# Autodesk Inventor assembly: !drivetrain
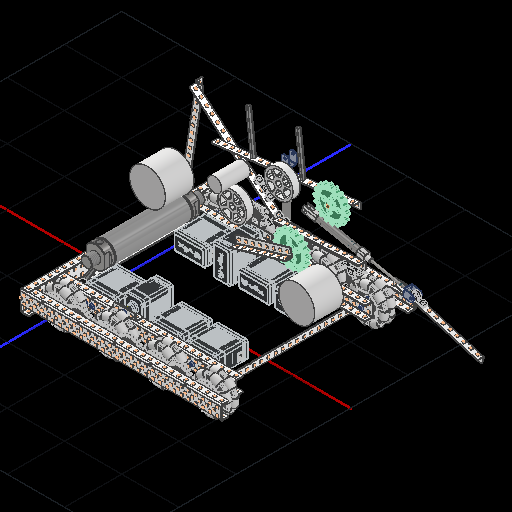
[picture p0: Inventor's stored thumbnail of the model, 512x512]
Saved by Autodesk Inventor 2025.2 (Build 292293000, 293)
## iProperties
Created: 2025-11-15
Part Number: !drivetrain
Document SubType Name: Assembly
Designer: cloudy
Author: cloudy
## Documents named in this file (43)
- C:\Users\cloudy\Documents\AURA_CAD\15\Drivetrain\!drivetrain.iam
- C:\Users\cloudy\Documents\AURA_CAD\15\Drivetrain\Wheels\Omni\2.75\2.75 Omni Assembly.iam
- C:\Users\cloudy\Documents\AURA_CAD\!lib\Structure\C Channel\Aluminum 1x2x1\Alu C 1x2x1x28.ipt
- C:\Users\cloudy\Documents\AURA_CAD\!lib\Structure\Hardware\Screw Steel - Star\SScrew Star Smooth 2.000.ipt
- C:\Users\cloudy\Documents\AURA_CAD\!lib\Structure\Hardware\Screw Steel - Star.ipt
- C:\Users\cloudy\Documents\AURA_CAD\!lib\Structure\Hardware\Nut Keps.ipt
- C:\Users\cloudy\Documents\AURA_CAD\!lib\Motion\Shaft LS\LS Pillow Bearing Block.ipt
- C:\Users\cloudy\Documents\AURA_CAD\!lib\Structure\C Channel\Aluminum 1x3x1 Half\Alu C Half 1x3x1x19.ipt
- C:\Users\cloudy\Documents\AURA_CAD\!lib\Structure\C Channel\Aluminum 1x2x1\Alu C 1x2x1x26.ipt
- C:\Users\cloudy\Documents\AURA_CAD\!lib\Structure\C Channel\Aluminum 1x3x1\Alu C 1x3x1x27.ipt
- C:\Users\cloudy\Documents\AURA_CAD\15\Drivetrain\Gears\26t_no_screwholes.ipt
- C:\Users\cloudy\Documents\AURA_CAD\!lib\Electronics\Motors with Screws\AluM-StarS.iam
- C:\Users\cloudy\Documents\AURA_CAD\!lib\Electronics\Motors with Screws.iam
- C:\Users\cloudy\Documents\AURA_CAD\15\Drivetrain\bearing_2 long.ipt
- C:\Users\cloudy\Documents\AURA_CAD\!lib\Motion\Spacers\Spacer Nylon .500 OD\NSpacer White .500 OD x .125.ipt
- C:\Users\cloudy\Documents\AURA_CAD\!lib\Motion\Spacers\Spacer Nylon .500 OD.ipt
- C:\Users\cloudy\Documents\AURA_CAD\!lib\Motion\Spacers\Spacer Nylon .375 OD\NSpacer .375 OD x .500.ipt
- C:\Users\cloudy\Documents\AURA_CAD\!lib\Motion\Spacers\Spacer Nylon .375 OD.ipt
- C:\Users\cloudy\Documents\AURA_CAD\!lib\Motion\Spacers\Spacer Nylon .375 OD\NSpacer .375 OD x .250.ipt
- C:\Users\cloudy\Documents\AURA_CAD\!lib\Motion\Shaft LS\Bearing Flat - Drilled.ipt
- C:\Users\cloudy\Documents\AURA_CAD\!lib\Motion\Shaft LS\Shaft Collar Metal\Shaft Collar No Screw.iam
- C:\Users\cloudy\Documents\AURA_CAD\!lib\Motion\Shaft LS\Shaft Collar Metal.iam
- C:\Users\cloudy\Documents\AURA_CAD\!lib\Structure\Standoff\Standoff 3.00.ipt
- C:\Users\cloudy\Documents\AURA_CAD\!lib\Structure\Standoff.ipt
- C:\Users\cloudy\Documents\AURA_CAD\!lib\Motion\Spacers\Spacer Nylon .375 OD\NSpacer .375 OD x .375.ipt
- C:\Users\cloudy\Documents\AURA_CAD\!lib\Motion\Spacers\Washer Steel\SWasher .375 OD x .062500.ipt
- C:\Users\cloudy\Documents\AURA_CAD\!lib\Motion\Spacers\Washer Steel.ipt
- C:\Users\cloudy\Documents\AURA_CAD\!lib\Structure\C Channel\Aluminum 1x3x1 Half\Alu C Half 1x3x1x3.ipt
- C:\Users\cloudy\Documents\AURA_CAD\!lib\Structure\C Channel\Aluminum 1x3x1 Half\Alu C Half 1x3x1x20.ipt
- C:\Users\cloudy\Documents\AURA_CAD\!lib\Motion\Pneumatics\Legacy - SMC Pneumatics\Double Acting Piston.iam
- C:\Users\cloudy\Documents\AURA_CAD\!lib\Motion\Pneumatics\Legacy - SMC Pneumatics\Cylinder Mount.ipt
- C:\Users\cloudy\Documents\AURA_CAD\!lib\Structure\C Channel\Aluminum 1x3x1 Half\Alu C Half 1x3x1x23.ipt
- C:\Users\cloudy\Documents\AURA_CAD\!lib\Structure\C Channel\Aluminum 1x3x1 Half\Alu C Half 1x3x1x15.ipt
- C:\Users\cloudy\Documents\AURA_CAD\!lib\Motion\Sprockets\9P Sprocket.iam
- C:\Users\cloudy\Documents\AURA_CAD\!lib\Motion\Sprockets\9P Sprocket\9P 18T Sprocket, Circle.iam
- C:\Users\cloudy\Documents\AURA_CAD\15\2.5in roller.ipt
- C:\Users\cloudy\Documents\AURA_CAD\!lib\Motion\Wheels\Flex Wheels\2.000 Flex Wheel\2.000 30A .500.ipt
- C:\Users\cloudy\Documents\AURA_CAD\!lib\Motion\Wheels\Flex Wheels\2.000 Flex Wheel.ipt
- C:\Users\cloudy\Documents\AURA_CAD\15\1 in roller.ipt
- C:\Users\cloudy\Documents\AURA_CAD\!lib\Motion\Pneumatics\Legacy - SMC Pneumatics\Reservoir.ipt
- C:\Users\cloudy\Documents\AURA_CAD\!lib\Structure\C Channel\Aluminum 1x3x1 Half\Alu C Half 1x3x1x8.ipt
- C:\Users\cloudy\Documents\AURA_CAD\!lib\Structure\C Channel\Aluminum 1x3x1 Half\Alu C Half 1x3x1x12.ipt
- C:\Users\cloudy\Documents\AURA_CAD\!lib\Structure\C Channel\Aluminum 1x3x1 Half\Alu C Half 1x3x1x2.ipt
## Components (111 placed, 33 different names)
1. Alu C 1x2x1x26:1 — Insert:10, Insert:19, Insert:20, Insert:23, Insert:26, Mate:18, Insert:36, Insert:40, Mate:22, Mate:23, Insert:41, Insert:42, Insert:43, Insert:47, Mate:24, Insert:51, Insert:67, Insert:90, Mate:37, Mate:38, Insert:102, Mate:44, Insert:112, Angle:1
2. 2.75 Omni Assembly:1 [sub-assembly] — Insert:45
3. Alu C 1x2x1x28:2 — Mate:17, Insert:33
4. Alu C 1x2x1x26:2 — Mate:14, Mate:18, Insert:31, Insert:93, Mate:39
5. SScrew Star Smooth 2.000:1 — Insert:10, Mate:26
6. 2.75 Omni Assembly:5 [sub-assembly] — Insert:46
7. SScrew Star Smooth 2.000:2 — Insert:20
8. 2.75 Omni Assembly:6 [sub-assembly] — Insert:23
9. SScrew Star Smooth 2.000:3 — Insert:19
10. 2.75 Omni Assembly:7 [sub-assembly] — Insert:44
11. Alu C Half 1x3x1x19:1 — Insert:26, Insert:31
12. Alu C 1x3x1x27:1 — Mate:14, Mate:15, Mate:16, Mate:17, Insert:32, Insert:33, Mate:34, Insert:72, Insert:108
13. 26t_no_screwholes:1 — Insert:52, Insert:56
14. 26t_no_screwholes:2 — Insert:53, Insert:55
15. 26t_no_screwholes:3 — Insert:54, Insert:57
16. Alu C 1x2x1x28:3 — Insert:32, Mate:26, Insert:52, Insert:53, Insert:54, Insert:58, Insert:59, Insert:60, Mate:27, Mate:28, Mate:29, Insert:61, Mate:30, Insert:62, Insert:63, Insert:64, Mate:31, Mate:32, Mate:33, Insert:130, Mate:57
17. AluM-StarS:1 [sub-assembly] — Insert:36, Mate:22
18. AluM-StarS:2 [sub-assembly] — Insert:40, Mate:23
19. AluM-StarS:3 [sub-assembly] — Insert:47, Mate:24
20. Nut Keps:1 — Insert:41, Insert:44
21. Nut Keps:2 — Insert:42, Insert:45
22. Nut Keps:3 — Insert:43, Insert:46
23. NSpacer White .500 OD x .125:2 — Insert:51
24. NSpacer .375 OD x .250:2 — Insert:56
25. NSpacer .375 OD x .250:3 — Insert:55
26. NSpacer .375 OD x .250:4 — Insert:57
27. bearing_2 long:3 — Insert:59, Mate:28
28. bearing_2 long:4 — Insert:61, Mate:30
29. bearing_2 long:5 — Insert:58, Mate:29
30. bearing_2 long:6 — Insert:60, Mate:27
31. Bearing Flat - Drilled:1 — Insert:62, Mate:33
32. Bearing Flat - Drilled:2 — Insert:64, Mate:31
33. Bearing Flat - Drilled:3 — Insert:63, Mate:32
34. Shaft Collar No Screw:1 [sub-assembly] — Insert:67, Mate:35, Insert:69
35. Shaft Collar No Screw:2 [sub-assembly] — Mate:34, Mate:35, Insert:68, Insert:74
36. Standoff 3.00:1 — Insert:70
37. NSpacer .375 OD x .500:5 — Insert:68
38. NSpacer .375 OD x .375:6 — Insert:69, Insert:70
39. NSpacer .375 OD x .500:7 — Insert:71, Insert:73
40. NSpacer .375 OD x .500:8 — Insert:71, Insert:72
41. SWasher .375 OD x .062500:1 — Insert:73
42. SWasher .375 OD x .062500:2 — Insert:74
43. 2.75 Omni Assembly:8 [sub-assembly] — Insert:76
44. SScrew Star Smooth 2.000:6
45. 2.75 Omni Assembly:9 [sub-assembly] — Insert:77
46. SScrew Star Smooth 2.000:7
47. 2.75 Omni Assembly:10 [sub-assembly]
48. SScrew Star Smooth 2.000:8
49. 2.75 Omni Assembly:11 [sub-assembly] — Insert:75
50. 26t_no_screwholes:4 — Insert:80
51. 26t_no_screwholes:5 — Insert:81
52. 26t_no_screwholes:6 — Insert:82
53. AluM-StarS:4 [sub-assembly]
54. AluM-StarS:5 [sub-assembly]
55. AluM-StarS:6 [sub-assembly]
56. Nut Keps:4 — Insert:75
57. Nut Keps:5 — Insert:76
58. Nut Keps:6 — Insert:77
59. NSpacer White .500 OD x .125:4
60. NSpacer .375 OD x .250:10 — Insert:80
61. NSpacer .375 OD x .250:11 — Insert:81
62. NSpacer .375 OD x .250:12 — Insert:82
63. bearing_2 long:7
64. bearing_2 long:8
65. bearing_2 long:9
66. bearing_2 long:10
67. Bearing Flat - Drilled:4
68. Bearing Flat - Drilled:5
69. Bearing Flat - Drilled:6
70. Shaft Collar No Screw:3 [sub-assembly] — Mate:36, Insert:86
71. Shaft Collar No Screw:4 [sub-assembly] — Mate:36, Insert:84, Insert:89
72. Standoff 3.00:2 — Insert:85
73. NSpacer .375 OD x .500:13 — Insert:84
74. NSpacer .375 OD x .375:14 — Insert:85, Insert:86
75. NSpacer .375 OD x .500:15 — Insert:87, Insert:88
76. NSpacer .375 OD x .500:16 — Insert:87
77. SWasher .375 OD x .062500:3 — Insert:88
78. SWasher .375 OD x .062500:4 — Insert:89
79. Alu C Half 1x3x1x3:1 — Insert:90, Mate:37, Insert:91
80. AluM-StarS:7 [sub-assembly] — Insert:91, Mate:38
81. Alu C Half 1x3x1x3:2 — Insert:92, Insert:93, Mate:39
82. AluM-StarS:8 [sub-assembly] — Insert:92
83. Alu C Half 1x3x1x23:1 — Mate:48, Insert:110, Insert:121, Mate:53, Insert:123, Mate:54, Insert:126, Mate:55, Mate:138
84. LS Pillow Bearing Block:2 — Insert:102, Mate:44
85. Shaft Collar No Screw:5 [sub-assembly] — Insert:108, Insert:109
86. Alu C Half 1x3x1x15:1 — Insert:109, Mate:48
87. Alu C Half 1x3x1x20:1 — Insert:110, Insert:111, Mate:51, Mate:52, Insert:115, Insert:116, Insert:117, Insert:118
88. 9P 18T Sprocket, Circle:1 [sub-assembly] — Insert:111
89. 2.5in roller:1 — Mate:51
90. Shaft Collar No Screw:6 [sub-assembly] — Insert:112, Insert:113
91. Double Acting Piston:1 [sub-assembly] — Insert:113, Insert:114, Angle:1
92. Cylinder Mount:1 — Insert:114, Mate:52
93. Standoff 3.00:3 — Insert:115
94. Standoff 3.00:4 — Insert:116
95. 2.000 30A .500:1 — Insert:117
96. 1 in roller:1 — Insert:118
97. 2.5in roller:2 — Insert:129
98. 9P 18T Sprocket, Circle:2 [sub-assembly] — Insert:125
99. 2.000 30A .500:2 — Insert:122
100. Reservoir:1
101. LS Pillow Bearing Block:3 — Insert:121, Mate:53, Insert:122
102. LS Pillow Bearing Block:4 — Insert:123, Mate:54, Insert:124
103. Alu C Half 1x3x1x8:1 — Insert:124, Insert:125
104. LS Pillow Bearing Block:5 — Insert:126, Mate:55, Insert:127
105. Alu C Half 1x3x1x12:1 — Insert:127, Insert:128, Mate:56
106. LS Pillow Bearing Block:6 — Insert:128, Mate:56, Insert:129
107. Alu C Half 1x3x1x2:1 — Insert:130, Mate:57, Insert:131
108. Alu C Half 1x3x1x12:2 — Insert:131, Insert:134, Mate:139
109. Double Acting Piston:2 [sub-assembly] — Mate:138
110. Cylinder Mount:2 — Insert:133
111. LS Pillow Bearing Block:7 — Insert:133, Insert:134, Mate:139
## Relationships (117: Insert 82, Mate 34, Angle 1)
- [Mate]: Alu C 1x2x1x28:2 ↔ Alu C 1x2x1x26:2
- Insert:10: Alu C 1x2x1x26:1 ↔ SScrew Star Smooth 2.000:1
- Insert:19: Alu C 1x2x1x26:1 ↔ SScrew Star Smooth 2.000:3
- Insert:20: Alu C 1x2x1x26:1 ↔ SScrew Star Smooth 2.000:2
- Insert:23 (4.191 mm): Alu C 1x2x1x26:1 ↔ 2.75 Omni Assembly:6
- Insert:26 (12.7 mm): Alu C 1x2x1x26:1 ↔ Alu C Half 1x3x1x19:1
- Mate:14: Alu C 1x2x1x26:2 ↔ Alu C 1x3x1x27:1
- Mate:15: Alu C 1x3x1x27:1
- Mate:16: Alu C 1x3x1x27:1
- Mate:17: Alu C 1x2x1x28:2 ↔ Alu C 1x3x1x27:1
- Mate:18: Alu C 1x2x1x26:1 ↔ Alu C 1x2x1x26:2
- Insert:31 (12.7 mm): Alu C 1x2x1x26:2 ↔ Alu C Half 1x3x1x19:1
- Insert:32: Alu C 1x3x1x27:1 ↔ Alu C 1x2x1x28:3
- Insert:33: Alu C 1x2x1x28:2 ↔ Alu C 1x3x1x27:1
- Insert:36: Alu C 1x2x1x26:1 ↔ AluM-StarS:1
- Insert:40: Alu C 1x2x1x26:1 ↔ AluM-StarS:2
- Mate:22: Alu C 1x2x1x26:1 ↔ AluM-StarS:1
- Mate:23: Alu C 1x2x1x26:1 ↔ AluM-StarS:2
- Insert:41: Alu C 1x2x1x26:1 ↔ Nut Keps:1
- Insert:42: Alu C 1x2x1x26:1 ↔ Nut Keps:2
- Insert:43: Alu C 1x2x1x26:1 ↔ Nut Keps:3
- Insert:44 (0.7937 mm): 2.75 Omni Assembly:7 ↔ Nut Keps:1
- Insert:45 (0.7937 mm): 2.75 Omni Assembly:1 ↔ Nut Keps:2
- Insert:46 (0.7937 mm): 2.75 Omni Assembly:5 ↔ Nut Keps:3
- Insert:47: Alu C 1x2x1x26:1 ↔ AluM-StarS:3
- Mate:24: Alu C 1x2x1x26:1 ↔ AluM-StarS:3
- Insert:51: Alu C 1x2x1x26:1 ↔ NSpacer White .500 OD x .125:2
- Mate:26: SScrew Star Smooth 2.000:1 ↔ Alu C 1x2x1x28:3
- Insert:52 (13.4938 mm): 26t_no_screwholes:1 ↔ Alu C 1x2x1x28:3
- Insert:53 (13.4938 mm): 26t_no_screwholes:2 ↔ Alu C 1x2x1x28:3
- Insert:54 (13.4938 mm): 26t_no_screwholes:3 ↔ Alu C 1x2x1x28:3
- Insert:55: 26t_no_screwholes:2 ↔ NSpacer .375 OD x .250:3
- Insert:56: 26t_no_screwholes:1 ↔ NSpacer .375 OD x .250:2
- Insert:57: 26t_no_screwholes:3 ↔ NSpacer .375 OD x .250:4
- Insert:58: Alu C 1x2x1x28:3 ↔ bearing_2 long:5
- Insert:59: Alu C 1x2x1x28:3 ↔ bearing_2 long:3
- Insert:60: Alu C 1x2x1x28:3 ↔ bearing_2 long:6
- Mate:27: Alu C 1x2x1x28:3 ↔ bearing_2 long:6
- Mate:28: Alu C 1x2x1x28:3 ↔ bearing_2 long:3
- Mate:29: Alu C 1x2x1x28:3 ↔ bearing_2 long:5
- Insert:61: Alu C 1x2x1x28:3 ↔ bearing_2 long:4
- Mate:30: Alu C 1x2x1x28:3 ↔ bearing_2 long:4
- Insert:62: Alu C 1x2x1x28:3 ↔ Bearing Flat - Drilled:1
- Insert:63: Alu C 1x2x1x28:3 ↔ Bearing Flat - Drilled:3
- Insert:64: Alu C 1x2x1x28:3 ↔ Bearing Flat - Drilled:2
- Mate:31: Alu C 1x2x1x28:3 ↔ Bearing Flat - Drilled:2
- Mate:32: Alu C 1x2x1x28:3 ↔ Bearing Flat - Drilled:3
- Mate:33: Alu C 1x2x1x28:3 ↔ Bearing Flat - Drilled:1
- Insert:67: Alu C 1x2x1x26:1 ↔ Shaft Collar No Screw:1
- Mate:34: Alu C 1x3x1x27:1 ↔ Shaft Collar No Screw:2
- Mate:35: Shaft Collar No Screw:1 ↔ Shaft Collar No Screw:2
- Insert:68: Shaft Collar No Screw:2 ↔ NSpacer .375 OD x .500:5
- Insert:69: Shaft Collar No Screw:1 ↔ NSpacer .375 OD x .375:6
- Insert:70: Standoff 3.00:1 ↔ NSpacer .375 OD x .375:6
- Insert:71: NSpacer .375 OD x .500:7 ↔ NSpacer .375 OD x .500:8
- Insert:72: Alu C 1x3x1x27:1 ↔ NSpacer .375 OD x .500:8
- Insert:73: NSpacer .375 OD x .500:7 ↔ SWasher .375 OD x .062500:1
- Insert:74: Shaft Collar No Screw:2 ↔ SWasher .375 OD x .062500:2
- Insert:75 (0.7937 mm): 2.75 Omni Assembly:11 ↔ Nut Keps:4
- Insert:76 (0.7937 mm): 2.75 Omni Assembly:8 ↔ Nut Keps:5
- Insert:77 (0.7937 mm): 2.75 Omni Assembly:9 ↔ Nut Keps:6
- Insert:80: 26t_no_screwholes:4 ↔ NSpacer .375 OD x .250:10
- Insert:81: 26t_no_screwholes:5 ↔ NSpacer .375 OD x .250:11
- Insert:82: 26t_no_screwholes:6 ↔ NSpacer .375 OD x .250:12
- Mate:36: Shaft Collar No Screw:3 ↔ Shaft Collar No Screw:4
- Insert:84: Shaft Collar No Screw:4 ↔ NSpacer .375 OD x .500:13
- Insert:85: Standoff 3.00:2 ↔ NSpacer .375 OD x .375:14
- Insert:86: Shaft Collar No Screw:3 ↔ NSpacer .375 OD x .375:14
- Insert:87: NSpacer .375 OD x .500:15 ↔ NSpacer .375 OD x .500:16
- Insert:88: NSpacer .375 OD x .500:15 ↔ SWasher .375 OD x .062500:3
- Insert:89: Shaft Collar No Screw:4 ↔ SWasher .375 OD x .062500:4
- Insert:90: Alu C 1x2x1x26:1 ↔ Alu C Half 1x3x1x3:1
- Mate:37: Alu C 1x2x1x26:1 ↔ Alu C Half 1x3x1x3:1
- Insert:91: Alu C Half 1x3x1x3:1 ↔ AluM-StarS:7
- Mate:38: Alu C 1x2x1x26:1 ↔ AluM-StarS:7
- Insert:92: Alu C Half 1x3x1x3:2 ↔ AluM-StarS:8
- Insert:93: Alu C 1x2x1x26:2 ↔ Alu C Half 1x3x1x3:2
- Mate:39: Alu C 1x2x1x26:2 ↔ Alu C Half 1x3x1x3:2
- [Insert] (3.175 mm): Alu C Half 1x3x1x23:1 ↔ LS Pillow Bearing Block:2
- Insert:102: Alu C 1x2x1x26:1 ↔ LS Pillow Bearing Block:2
- Mate:44: Alu C 1x2x1x26:1 ↔ LS Pillow Bearing Block:2
- Insert:108 (3.175 mm): Alu C 1x3x1x27:1 ↔ Shaft Collar No Screw:5
- Insert:109: Shaft Collar No Screw:5 ↔ Alu C Half 1x3x1x15:1
- Mate:48: Alu C Half 1x3x1x23:1 ↔ Alu C Half 1x3x1x15:1
- Insert:110 (12.7 mm): Alu C Half 1x3x1x23:1 ↔ Alu C Half 1x3x1x20:1
- Insert:111 (12.7 mm): Alu C Half 1x3x1x20:1 ↔ 9P 18T Sprocket, Circle:1
- Mate:51: Alu C Half 1x3x1x20:1 ↔ 2.5in roller:1
- Insert:112: Alu C 1x2x1x26:1 ↔ Shaft Collar No Screw:6
- Insert:113: Shaft Collar No Screw:6 ↔ Double Acting Piston:1
- Insert:114 (-5.08 mm): Double Acting Piston:1 ↔ Cylinder Mount:1
- Mate:52: Alu C Half 1x3x1x20:1 ↔ Cylinder Mount:1
- Insert:115: Alu C Half 1x3x1x20:1 ↔ Standoff 3.00:3
- Insert:116: Alu C Half 1x3x1x20:1 ↔ Standoff 3.00:4
- Insert:117 (12.7 mm): Alu C Half 1x3x1x20:1 ↔ 2.000 30A .500:1
- Insert:118 (25.4 mm): Alu C Half 1x3x1x20:1 ↔ 1 in roller:1
- Insert:121 (6.35 mm): Alu C Half 1x3x1x23:1 ↔ LS Pillow Bearing Block:3
- Mate:53: Alu C Half 1x3x1x23:1 ↔ LS Pillow Bearing Block:3
- Angle:1 (0 deg): Alu C 1x2x1x26:1 ↔ Double Acting Piston:1
- Insert:122 (50.8 mm): 2.000 30A .500:2 ↔ LS Pillow Bearing Block:3
- Insert:123 (12.7 mm): Alu C Half 1x3x1x23:1 ↔ LS Pillow Bearing Block:4
- Mate:54: Alu C Half 1x3x1x23:1 ↔ LS Pillow Bearing Block:4
- Insert:124 (50.8 mm): LS Pillow Bearing Block:4 ↔ Alu C Half 1x3x1x8:1
- Insert:125: 9P 18T Sprocket, Circle:2 ↔ Alu C Half 1x3x1x8:1
- Insert:126: Alu C Half 1x3x1x23:1 ↔ LS Pillow Bearing Block:5
- Mate:55: Alu C Half 1x3x1x23:1 ↔ LS Pillow Bearing Block:5
- Insert:127: LS Pillow Bearing Block:5 ↔ Alu C Half 1x3x1x12:1
- Insert:128 (12.7 mm): Alu C Half 1x3x1x12:1 ↔ LS Pillow Bearing Block:6
- Mate:56: Alu C Half 1x3x1x12:1 ↔ LS Pillow Bearing Block:6
- Insert:129 (50.8 mm): 2.5in roller:2 ↔ LS Pillow Bearing Block:6
- Insert:130 (3.175 mm): Alu C 1x2x1x28:3 ↔ Alu C Half 1x3x1x2:1
- Mate:57: Alu C 1x2x1x28:3 ↔ Alu C Half 1x3x1x2:1
- Insert:131: Alu C Half 1x3x1x2:1 ↔ Alu C Half 1x3x1x12:2
- [Insert] (-5.08 mm): Double Acting Piston:2 ↔ Cylinder Mount:2
- Insert:133: Cylinder Mount:2 ↔ LS Pillow Bearing Block:7
- Mate:138: Alu C Half 1x3x1x23:1 ↔ Double Acting Piston:2
- Insert:134: Alu C Half 1x3x1x12:2 ↔ LS Pillow Bearing Block:7
- Mate:139: Alu C Half 1x3x1x12:2 ↔ LS Pillow Bearing Block:7
## Named parameters: d9_d5 = 0 mm, d164_d162 = 3.175 mm, d236_d202 = -5.08 mm
